# Autodesk Inventor assembly: one roller asmb
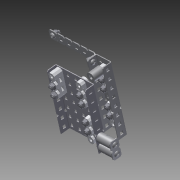
[picture p0: Inventor's stored thumbnail of the model, 180x180]
Saved by Autodesk Inventor 2014 SP1 (Build 180222100, 222)
## iProperties
Created: 2014-03-20
Part Number: one roller asmb
Document SubType Name: Assembly
Designer: Ryan
Author: Ryan
## Documents named in this file (15)
- C:\Users\Ryan\Desktop\sw\toss up 5th A bot\intake\6 bar attachment.iam
- C:\Users\Ryan\Desktop\sw\lib\Aperture VEX CAD Library\Hardware\8-32\8-32 nylock.ipt
- C:\Users\Ryan\Desktop\sw\lib\Aperture VEX CAD Library\Bearing Blocks\Bearing Block.ipt
- C:\Users\Ryan\Desktop\sw\lib\Aperture VEX CAD Library\Metal\C Channel\5 x 7.ipt
- C:\Users\Ryan\Desktop\sw\lib\Aperture VEX CAD Library\Hardware\8-32\8-32_.500.ipt
- C:\Users\Ryan\Desktop\sw\lib\Aperture VEX CAD Library\Metal\C Channel\2 x 8.ipt
- C:\Users\Ryan\Desktop\sw\lib\Aperture VEX CAD Library\Hardware\8-32\8-23_.750.ipt
- C:\Users\Ryan\Desktop\sw\lib\Aperture VEX CAD Library\Spacers\SPACER-0500-0375.ipt
- C:\Users\Ryan\Desktop\sw\lib\Aperture VEX CAD Library\Spacers\SPACER-0500-0250.ipt
- C:\Users\Ryan\Desktop\sw\lib\Aperture VEX CAD Library\Spacers\SPACER-0500-0125.ipt
- C:\Users\Ryan\Desktop\sw\lib\Aperture VEX CAD Library\Hardware\8-32\8-32_.375.ipt
- C:\Users\Ryan\Desktop\sw\lib\Aperture VEX CAD Library\Metal\Custom 1 bar\6 bend 1.ipt
- C:\Users\Ryan\Desktop\sw\lib\Aperture VEX CAD Library\Spacers\SPACER-0500-0500.ipt
- C:\Users\Ryan\Desktop\sw\lib\Aperture VEX CAD Library\Hardware\8-32\8-32_1.000.ipt
- C:\Users\Ryan\Desktop\sw\lib\Aperture VEX CAD Library\Metal\Custom 1 bar\1x2 bar.ipt
## Components (45 placed, 14 different names)
1. 5 x 7:1 — Mate:66, Mate:67, Mate:70, Mate:73, Mate:74, Mate:75, Mate:76, Mate:77, Mate:78, Mate:79, Mate:80, Mate:81, Mate:83, Flush:2, Flush:3, Mate:88, Mate:90, Mate:99, Mate:118, Mate:119, Mate:120, Flush:5, Flush:6, Mate:126
2. Bearing Block:4 — Mate:66, Mate:74, Mate:75, Mate:89
3. Bearing Block:5 — Mate:67, Mate:87, Mate:92, Mate:94
4. 2 x 8:1 — Flush:2, Flush:3, Mate:86, Mate:102, Mate:103, Mate:104, Mate:106, Flush:4
5. 8-23_.750:1 — Mate:87, Mate:88, Mate:91
6. 8-23_.750:2 — Mate:89, Mate:90, Mate:93
7. 8-32 nylock:16 — Mate:91, Mate:92
8. 8-32 nylock:17 — Mate:93, Mate:94
9. SPACER-0500-0375:1 — Mate:95, Mate:96, Mate:101
10. SPACER-0500-0250:1 — Mate:95, Mate:96, Mate:98
11. SPACER-0500-0125:1 — Mate:99, Mate:100, Mate:101
12. 8-32_.375:1 — Mate:102, Mate:103, Mate:104, Mate:105, Mate:107, Mate:108
13. 8-32 nylock:18 — Mate:105, Mate:109
14. 6 bend 1:1 — Mate:106, Mate:107, Mate:108, Mate:109, Flush:4, Mate:110, Mate:111, Mate:112, Mate:114
15. 8-32_.375:2 — Mate:110, Mate:111, Mate:112, Mate:113
16. 8-32 nylock:19 — Mate:113, Mate:114
17. 1x2 bar:1 — Mate:124, Flush:5, Flush:6, Mate:125
18. Bearing Block:6 — Mate:70, Mate:73, Mate:76, Mate:77, Mate:82, Mate:85, Mate:100
19. Bearing Block:7 — Mate:78, Mate:79, Mate:80, Mate:81
20. Bearing Block:8 — Mate:86, Mate:98
21. Bearing Block:9
22. SPACER-0500-0500:1 — Mate:121, Mate:122, Mate:123, Mate:124
23. SPACER-0500-0375:2 — Mate:118, Mate:119, Mate:120, Mate:121, Mate:122, Mate:127
24. 8-32_1.000:1 — Mate:123, Mate:125
25. 8-32 nylock:20 — Mate:126, Mate:127
26. SPACER-0500-0500:2
27. SPACER-0500-0375:3
28. 8-32_1.000:2
29. 8-32 nylock:21
30. 8-32_.500:1 — Mate:82, Mate:83, Mate:84
31. 8-32 nylock:8 — Mate:84, Mate:85
32. 8-32_.500:2
33. 8-32 nylock:9
34. 8-32_.500:3
35. 8-32 nylock:10
36. 8-32_.500:4
37. 8-32 nylock:11
38. 8-32_.500:5
39. 8-32 nylock:12
40. 8-32_.500:6
41. 8-32 nylock:13
42. 8-32_.500:7
43. 8-32 nylock:14
44. 8-32_.500:8
45. 8-32 nylock:15
## Component patterns: (2 elements, first: Bearing Block:6 + Bearing Block:7), (2 elements, first: SPACER-0500-0500:1 + SPACER-0500-0375:2 + 8-32_1.000:1 + 8-32 nylock:20), (4 elements, first: 8-32_.500:1 + 8-32 nylock:8), Component Pattern 1:2 (4 elements)
## Relationships (62: Mate 57, Flush 5)
- [Mate]: Bearing Block:4 ↔ Bearing Block:5
- [Mate]: Bearing Block:4 ↔ Bearing Block:5
- [Mate]: Bearing Block:4 ↔ Bearing Block:5
- Mate:66: 5 x 7:1 ↔ Bearing Block:4
- Mate:67 (2.3114 mm): 5 x 7:1 ↔ Bearing Block:5
- Mate:70: 5 x 7:1 ↔ Bearing Block:6
- Mate:73 (2.3114 mm): 5 x 7:1 ↔ Bearing Block:6
- Mate:74 (2.3114 mm): 5 x 7:1 ↔ Bearing Block:4
- Mate:75 (2.3114 mm): 5 x 7:1 ↔ Bearing Block:4
- Mate:76 (2.3114 mm): 5 x 7:1 ↔ Bearing Block:6
- Mate:77 (2.3114 mm): 5 x 7:1 ↔ Bearing Block:6
- Mate:78: 5 x 7:1 ↔ Bearing Block:7
- Mate:79 (2.3114 mm): 5 x 7:1 ↔ Bearing Block:7
- Mate:80 (2.3114 mm): 5 x 7:1 ↔ Bearing Block:7
- Mate:81 (2.3114 mm): 5 x 7:1 ↔ Bearing Block:7
- Mate:82: Bearing Block:6 ↔ 8-32_.500:1
- Mate:83: 5 x 7:1 ↔ 8-32_.500:1
- Mate:84: 8-32_.500:1 ↔ 8-32 nylock:8
- Mate:85: Bearing Block:6 ↔ 8-32 nylock:8
- Flush:2: 5 x 7:1 ↔ 2 x 8:1
- Flush:3: 5 x 7:1 ↔ 2 x 8:1
- Mate:86: 2 x 8:1 ↔ Bearing Block:8
- Mate:87: Bearing Block:5 ↔ 8-23_.750:1
- Mate:88: 5 x 7:1 ↔ 8-23_.750:1
- Mate:89: Bearing Block:4 ↔ 8-23_.750:2
- Mate:90: 5 x 7:1 ↔ 8-23_.750:2
- Mate:91: 8-23_.750:1 ↔ 8-32 nylock:16
- Mate:92: Bearing Block:5 ↔ 8-32 nylock:16
- Mate:93: 8-23_.750:2 ↔ 8-32 nylock:17
- Mate:94: Bearing Block:5 ↔ 8-32 nylock:17
- Mate:95: SPACER-0500-0375:1 ↔ SPACER-0500-0250:1
- Mate:96: SPACER-0500-0375:1 ↔ SPACER-0500-0250:1
- Mate:98: SPACER-0500-0250:1 ↔ Bearing Block:8
- Mate:99: 5 x 7:1 ↔ SPACER-0500-0125:1
- Mate:100: SPACER-0500-0125:1 ↔ Bearing Block:6
- Mate:101 (7.5184 mm): SPACER-0500-0375:1 ↔ SPACER-0500-0125:1
- Mate:102 (2.3114 mm): 2 x 8:1 ↔ 8-32_.375:1
- Mate:103: 2 x 8:1 ↔ 8-32_.375:1
- Mate:104 (2.3114 mm): 2 x 8:1 ↔ 8-32_.375:1
- Mate:105: 8-32_.375:1 ↔ 8-32 nylock:18
- Mate:106: 2 x 8:1 ↔ 6 bend 1:1
- Mate:107 (2.3114 mm): 8-32_.375:1 ↔ 6 bend 1:1
- Mate:108 (2.3114 mm): 8-32_.375:1 ↔ 6 bend 1:1
- Mate:109: 8-32 nylock:18 ↔ 6 bend 1:1
- Flush:4: 2 x 8:1 ↔ 6 bend 1:1
- Mate:110 (2.3114 mm): 6 bend 1:1 ↔ 8-32_.375:2
- Mate:111 (2.3114 mm): 6 bend 1:1 ↔ 8-32_.375:2
- Mate:112: 6 bend 1:1 ↔ 8-32_.375:2
- Mate:113: 8-32_.375:2 ↔ 8-32 nylock:19
- Mate:114 (1.1684 mm): 6 bend 1:1 ↔ 8-32 nylock:19
- Mate:118 (2.3114 mm): 5 x 7:1 ↔ SPACER-0500-0375:2
- Mate:119 (2.3114 mm): 5 x 7:1 ↔ SPACER-0500-0375:2
- Mate:120: 5 x 7:1 ↔ SPACER-0500-0375:2
- Mate:121: SPACER-0500-0500:1 ↔ SPACER-0500-0375:2
- Mate:122: SPACER-0500-0500:1 ↔ SPACER-0500-0375:2
- Mate:123: SPACER-0500-0500:1 ↔ 8-32_1.000:1
- Mate:124: 1x2 bar:1 ↔ SPACER-0500-0500:1
- Flush:5: 5 x 7:1 ↔ 1x2 bar:1
- Flush:6: 5 x 7:1 ↔ 1x2 bar:1
- Mate:125: 1x2 bar:1 ↔ 8-32_1.000:1
- Mate:126: 5 x 7:1 ↔ 8-32 nylock:20
- Mate:127: SPACER-0500-0375:2 ↔ 8-32 nylock:20
## Named parameters: q = 2.3114 mm, d70_d63 = 0 mm, d71_d64 = 0 mm, d72_d65 = 0 mm
